# Autodesk Inventor assembly: XEndBushingRight
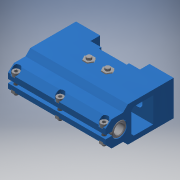
[picture p0: Inventor's stored thumbnail of the model, 180x180]
Saved by Autodesk Inventor 2016 (Build 200138000, 138)
## iProperties
Created: 2014-08-16
Part Number: XEndBushingRight
Document SubType Name: Assembly
Designer: Jack
Mass: 125.348 g
Surface Area: 370.67 cm^2
Volume: 71.2484 cm^3
Density: 1.75931 g/cm^3
Author: Jack
Title: X End Right
## Documents named in this file (13)
- C:\Users\Jack\ownCloud\Projects\CrossBot\InventorModel\XAxis\XEndBushingRight.iam
- C:\Users\Jack\ownCloud\Projects\CrossBot\InventorModel\Hardware\Nuts\Nut3.ipt
- C:\Users\Jack\ownCloud\Projects\CrossBot\InventorModel\Hardware\Bolts\SHCS\SHCS4\SHCS4x30.ipt
- C:\Users\Jack\ownCloud\Projects\CrossBot\InventorModel\Hardware\Nuts\Nut4.ipt
- C:\Users\Jack\ownCloud\Projects\CrossBot\InventorModel\Hardware\Bearing\BearingRadialBall\BearingRadialBallF624zz.ipt
- C:\Users\Jack\ownCloud\Projects\CrossBot\InventorModel\Hardware\Wahsers\M4Washer.ipt
- C:\Users\Jack\ownCloud\Projects\CrossBot\InventorModel\Hardware\Bolts\SHCS\SHCS3\SHCS3x8.ipt
- C:\Users\Jack\ownCloud\Projects\CrossBot\InventorModel\XAxis\XAxisBearingSpacer.ipt
- C:\Users\Jack\ownCloud\Projects\CrossBot\InventorModel\Hardware\Belt\GT2Idler.iam
- C:\Users\Jack\ownCloud\Projects\CrossBot\InventorModel\XAxis\XAxisBeltIdlerSpacer.ipt
- C:\Users\Jack\ownCloud\Projects\CrossBot\InventorModel\Hardware\Bolts\SHCS\SHCS3\SHCS3x14.ipt
- C:\Users\Jack\ownCloud\Projects\CrossBot\InventorModel\XAxis\XEndBushingRight.ipt
- C:\Users\Jack\ownCloud\Projects\CrossBot\InventorModel\Hardware\Bearing\BearingLinear\BearingLinearPlastic\BearingPlastic8x12x12.ipt
## Components (26 placed, 12 different names)
1. BearingRadialBallF624zz:1 — Mate:79, Mate:80, Mate:81, Mate:82
2. BearingRadialBallF624zz:2 — Mate:79, Mate:80, Mate:83
3. XAxisBearingSpacer:2 — Mate:84, Mate:85, Mate:138
4. GT2Idler:1 [sub-assembly] — Mate:86, Mate:121, Mate:137
5. XAxisBeltIdlerSpacer:1 — Mate:89, Mate:93, Mate:139
6. XEndBushingRight:1 — Mate:122, Mate:123, Mate:124, Mate:125, Mate:126, Mate:127, Mate:128, Mate:129, Angle:1, Angle:2, Angle:3, Mate:130, Mate:131, Mate:132, Angle:4, Mate:133, Mate:134, Mate:135, Angle:5, Mate:136, Mate:138, Mate:139, Mate:140, Mate:141, Angle:6, Angle:7, Mate:142, Mate:143, Mate:144, Mate:145, Flush:3, Flush:4
7. BearingPlastic8x12x12:1 — Mate:144, Flush:4
8. BearingPlastic8x12x12:2 — Mate:145, Flush:3
9. M4Washer:4 — Mate:38, Mate:137
10. M4Washer:3 — Mate:65, Mate:93, Mate:121
11. M4Washer:2 — Mate:30, Mate:82
12. M4Washer:1 — Mate:64, Mate:83, Mate:85
13. Nut4:2 — Mate:21, Angle:4, Mate:133
14. Nut4:1 — Mate:20, Angle:5, Mate:136
15. SHCS4x30:2 — Mate:20, Mate:38, Mate:65, Mate:86, Mate:89, Mate:134, Mate:135
16. SHCS4x30:1 — Mate:21, Mate:30, Mate:64, Mate:81, Mate:84, Mate:131, Mate:132
17. Nut3:3 — Mate:43, Angle:7, Mate:142, Flush:1
18. Nut3:4 — Mate:42, Angle:6, Mate:143, Flush:2
19. SHCS3x8:1 — Mate:42, Mate:141, Flush:2
20. SHCS3x8:2 — Mate:43, Mate:140, Flush:1
21. SHCS3x14:2 — Mate:111, Mate:124, Mate:125
22. Nut3:2 — Mate:111, Angle:2, Mate:130
23. SHCS3x14:3 — Mate:123, Mate:126
24. Nut3:5 — Mate:129, Angle:1
25. SHCS3x14:1 — Mate:114, Mate:122, Mate:127
26. Nut3:1 — Mate:114, Mate:128, Angle:3
## Relationships (57: Mate 46, Angle 7, Flush 4)
- Mate:20: Nut4:1 ↔ SHCS4x30:2
- Mate:21: Nut4:2 ↔ SHCS4x30:1
- Mate:30: M4Washer:2 ↔ SHCS4x30:1
- Mate:38: M4Washer:4 ↔ SHCS4x30:2
- Mate:42: Nut3:4 ↔ SHCS3x8:1
- Mate:43: Nut3:3 ↔ SHCS3x8:2
- Mate:64: M4Washer:1 ↔ SHCS4x30:1
- Mate:65: M4Washer:3 ↔ SHCS4x30:2
- Mate:79: BearingRadialBallF624zz:1 ↔ BearingRadialBallF624zz:2
- Mate:80: BearingRadialBallF624zz:1 ↔ BearingRadialBallF624zz:2
- Mate:81: BearingRadialBallF624zz:1 ↔ SHCS4x30:1
- Mate:82: BearingRadialBallF624zz:1 ↔ M4Washer:2
- Mate:83: BearingRadialBallF624zz:2 ↔ M4Washer:1
- Mate:84: XAxisBearingSpacer:2 ↔ SHCS4x30:1
- Mate:85: XAxisBearingSpacer:2 ↔ M4Washer:1
- Mate:86: GT2Idler:1 ↔ SHCS4x30:2
- Mate:89: XAxisBeltIdlerSpacer:1 ↔ SHCS4x30:2
- Mate:93: XAxisBeltIdlerSpacer:1 ↔ M4Washer:3
- Mate:111: SHCS3x14:2 ↔ Nut3:2
- Mate:114: SHCS3x14:1 ↔ Nut3:1
- [Mate]: SHCS3x14:3 ↔ Nut3:5
- Mate:121: GT2Idler:1 ↔ M4Washer:3
- Mate:122: XEndBushingRight:1 ↔ SHCS3x14:1
- Mate:123: XEndBushingRight:1 ↔ SHCS3x14:3
- Mate:124: XEndBushingRight:1 ↔ SHCS3x14:2
- Mate:125: XEndBushingRight:1 ↔ SHCS3x14:2
- Mate:126: XEndBushingRight:1 ↔ SHCS3x14:3
- Mate:127: XEndBushingRight:1 ↔ SHCS3x14:1
- Mate:128: XEndBushingRight:1 ↔ Nut3:1
- Mate:129: XEndBushingRight:1 ↔ Nut3:5
- Angle:1 (0 deg): XEndBushingRight:1 ↔ Nut3:5
- Angle:2 (0 deg): XEndBushingRight:1 ↔ Nut3:2
- Angle:3 (0 deg): XEndBushingRight:1 ↔ Nut3:1
- Mate:130: XEndBushingRight:1 ↔ Nut3:2
- Mate:131: XEndBushingRight:1 ↔ SHCS4x30:1
- Mate:132: XEndBushingRight:1 ↔ SHCS4x30:1
- Angle:4 (0 deg): XEndBushingRight:1 ↔ Nut4:2
- Mate:133: XEndBushingRight:1 ↔ Nut4:2
- Mate:134: XEndBushingRight:1 ↔ SHCS4x30:2
- Mate:135: XEndBushingRight:1 ↔ SHCS4x30:2
- Angle:5 (0 deg): XEndBushingRight:1 ↔ Nut4:1
- Mate:136: XEndBushingRight:1 ↔ Nut4:1
- Mate:137: GT2Idler:1 ↔ M4Washer:4
- Mate:138: XAxisBearingSpacer:2 ↔ XEndBushingRight:1
- Mate:139: XAxisBeltIdlerSpacer:1 ↔ XEndBushingRight:1
- Mate:140: XEndBushingRight:1 ↔ SHCS3x8:2
- Mate:141: XEndBushingRight:1 ↔ SHCS3x8:1
- Angle:6 (0 deg): XEndBushingRight:1 ↔ Nut3:4
- Angle:7 (0 deg): XEndBushingRight:1 ↔ Nut3:3
- Mate:142: XEndBushingRight:1 ↔ Nut3:3
- Mate:143: XEndBushingRight:1 ↔ Nut3:4
- Flush:1 (-0.5 mm): Nut3:3 ↔ SHCS3x8:2
- Flush:2 (-0.5 mm): Nut3:4 ↔ SHCS3x8:1
- Mate:144: XEndBushingRight:1 ↔ BearingPlastic8x12x12:1
- Mate:145: XEndBushingRight:1 ↔ BearingPlastic8x12x12:2
- Flush:3: XEndBushingRight:1 ↔ BearingPlastic8x12x12:2
- Flush:4: XEndBushingRight:1 ↔ BearingPlastic8x12x12:1
## Named parameters: d161_d150 = 0 mm
